# Autodesk Inventor assembly: ECoG holder
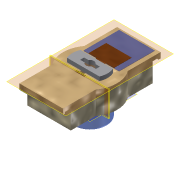
[picture p0: Inventor's stored thumbnail of the model, 180x180]
Saved by Autodesk Inventor 2014 (Build 180170000, 170)
## iProperties
Created: 2016-07-07
Part Number: ECoG holder
Document SubType Name: Assembly
Designer: Camilo
Author: Camilo
## Documents named in this file (8)
- Z:\Github\AgingTests\3D parts\ECoG holder\ECoG holder.iam
- Z:\Github\AgingTests\3D parts\ECoG holder\flaskPort.ipt
- Z:\Github\AgingTests\3D parts\ECoG holder\ECoG_holder.ipt
- Z:\Github\AgingTests\3D parts\ECoG holder\CoverSlip.ipt
- Z:\Github\AgingTests\3D parts\ECoG holder\ECoG64Ch.ipt
- Z:\Github\AgingTests\3D parts\ECoG holder\ECoG_holder_cap.ipt
- Z:\Github\AgingTests\3D parts\ECoG holder\coverSlip_5mmX10mm.ipt
- Z:\Github\AgingTests\3D parts\ECoG holder\ECoG_holder_cap2.ipt
## Components (8 placed, 7 different names)
1. flaskPort:1 — Flush:1
2. ECoG_holder:1 — Flush:1, Mate:1, Tangent:1, Mate:2, Flush:4, Flush:5, Mate:4, Mate:5, Mate:6, Mate:7, Mate:8, Mate:9, Flush:6, Flush:7
3. CoverSlip:1 — Mate:1, Tangent:1, Mate:2, Mate:3, Flush:2, Flush:3
4. ECoG64Ch:1 — Mate:3, Flush:2, Flush:3
5. ECoG_holder_cap:1 — Flush:4, Flush:5
6. coverSlip_5mmX10mm:1 — Mate:4, Mate:5, Mate:6
7. coverSlip_5mmX10mm:2 — Mate:7, Mate:8, Mate:9
8. ECoG_holder_cap2:1 — Flush:6, Flush:7
## Relationships (17: Mate 9, Flush 7, Tangent 1)
- Flush:1: flaskPort:1 ↔ ECoG_holder:1
- Mate:1: ECoG_holder:1 ↔ CoverSlip:1
- Tangent:1 (0.8 mm): ECoG_holder:1 ↔ CoverSlip:1
- Mate:2: ECoG_holder:1 ↔ CoverSlip:1
- Mate:3: CoverSlip:1 ↔ ECoG64Ch:1
- Flush:2: CoverSlip:1 ↔ ECoG64Ch:1
- Flush:3: CoverSlip:1 ↔ ECoG64Ch:1
- Flush:4: ECoG_holder:1 ↔ ECoG_holder_cap:1
- Flush:5: ECoG_holder:1 ↔ ECoG_holder_cap:1
- Mate:4: ECoG_holder:1 ↔ coverSlip_5mmX10mm:1
- Mate:5: ECoG_holder:1 ↔ coverSlip_5mmX10mm:1
- Mate:6: ECoG_holder:1 ↔ coverSlip_5mmX10mm:1
- Mate:7: ECoG_holder:1 ↔ coverSlip_5mmX10mm:2
- Mate:8: ECoG_holder:1 ↔ coverSlip_5mmX10mm:2
- Mate:9: ECoG_holder:1 ↔ coverSlip_5mmX10mm:2
- Flush:6: ECoG_holder:1 ↔ ECoG_holder_cap2:1
- Flush:7: ECoG_holder:1 ↔ ECoG_holder_cap2:1
